# Autodesk Inventor assembly: しゃーし
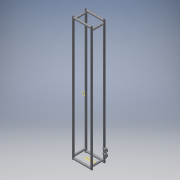
[picture p0: Inventor's stored thumbnail of the model, 180x180]
Saved by Autodesk Inventor 2018 (Build 220112000, 112)
## iProperties
Created: 2017-09-10
Part Number: しゃーし
Material: 一般
Document SubType Name: Assembly
Designer: Kenta
Author: Kenta
## Documents named in this file (7)
- C:\Users\Kenta\Documents\workspace\rbbr\cart\シャーシ\しゃーし.iam
- C:\Users\Kenta\Documents\workspace\rbbr\cart\シャーシ\横のパイプ.ipt
- C:\Users\Kenta\Documents\workspace\rbbr\cart\シャーシ\縦のパイプ.ipt
- C:\Users\Kenta\Documents\workspace\rbbr\cart\シャーシ\高さのパイプ.ipt
- C:\Users\Kenta\Documents\workspace\rbbr\cart\シャーシ\左右に飛び出すパイプ.ipt
- C:\Users\Kenta\Documents\workspace\rbbr\cart\シャーシ\14mmパイプ.ipt
- C:\Users\Kenta\Documents\workspace\rbbr\cart\シャーシ\hn1_14.ipt
## Components (17 placed, 6 different names)
1. 横のパイプ:1 — メイト:1, メイト:2, メイト:4, メイト:6, メイト:7, メイト:8, 角度:1
2. 縦のパイプ:1 — メイト:3, メイト:4, メイト:7, メイト:9, メイト:11, メイト:12, メイト:25, メイト:28, メイト:29, フラッシュ:3
3. 縦のパイプ:2 — メイト:5, メイト:6, メイト:8, メイト:10, メイト:21, メイト:23, メイト:27, メイト:30
4. 横のパイプ:2 — メイト:9, メイト:10, メイト:11
5. 高さのパイプ:1 — メイト:12, 角度:1, メイト:20, メイト:28
6. 横のパイプ:3
7. 縦のパイプ:3 — メイト:20, メイト:24, フラッシュ:3
8. 縦のパイプ:4 — メイト:22, メイト:26, メイト:31, メイト:33
9. 横のパイプ:4
10. 高さのパイプ:2 — メイト:24, メイト:25, メイト:29
11. 高さのパイプ:3 — メイト:23, メイト:26, メイト:30
12. 高さのパイプ:4 — メイト:21, メイト:22, メイト:27
13. 左右に飛び出すパイプ:1 — メイト:31, メイト:32, メイト:36
14. 14mmパイプ:1 — メイト:32, メイト:34, メイト:35, フラッシュ:4, メイト:37, フラッシュ:5
15. 左右に飛び出すパイプ:2 — メイト:33, メイト:34, メイト:38
16. hn1_14:1 — メイト:35, メイト:36, フラッシュ:4
17. hn1_14:2 — メイト:37, メイト:38, フラッシュ:5
## Relationships (44: Mate 38, Flush 5, Angle 1)
- フラッシュ:1 [Flush]
- メイト:1 [Mate]: 横のパイプ:1
- フラッシュ:2 [Flush]
- メイト:2 [Mate]: 横のパイプ:1
- メイト:3 [Mate]: 縦のパイプ:1
- メイト:4 [Mate]: 横のパイプ:1 ↔ 縦のパイプ:1
- メイト:5 [Mate]: 縦のパイプ:2
- メイト:6 [Mate]: 横のパイプ:1 ↔ 縦のパイプ:2
- メイト:7 [Mate] (-13.6 mm): 横のパイプ:1 ↔ 縦のパイプ:1
- メイト:8 [Mate] (-13.6 mm): 横のパイプ:1 ↔ 縦のパイプ:2
- メイト:9 [Mate]: 縦のパイプ:1 ↔ 横のパイプ:2
- メイト:10 [Mate]: 縦のパイプ:2 ↔ 横のパイプ:2
- メイト:11 [Mate] (-13.6 mm): 縦のパイプ:1 ↔ 横のパイプ:2
- メイト:12 [Mate]: 縦のパイプ:1 ↔ 高さのパイプ:1
- 角度:1 [Angle] (-90 deg): 横のパイプ:1 ↔ 高さのパイプ:1
- [Mate]: 横のパイプ:3 ↔ 縦のパイプ:3
- [Mate]: 横のパイプ:3 ↔ 縦のパイプ:4
- [Mate] (-13.6 mm): 横のパイプ:3 ↔ 縦のパイプ:3
- [Mate] (-13.6 mm): 横のパイプ:3 ↔ 縦のパイプ:4
- [Mate]: 縦のパイプ:3 ↔ 横のパイプ:4
- [Mate]: 縦のパイプ:4 ↔ 横のパイプ:4
- [Mate] (-13.6 mm): 縦のパイプ:3 ↔ 横のパイプ:4
- メイト:20 [Mate]: 高さのパイプ:1 ↔ 縦のパイプ:3
- メイト:21 [Mate]: 縦のパイプ:2 ↔ 高さのパイプ:4
- メイト:22 [Mate]: 縦のパイプ:4 ↔ 高さのパイプ:4
- メイト:23 [Mate]: 縦のパイプ:2 ↔ 高さのパイプ:3
- メイト:24 [Mate]: 縦のパイプ:3 ↔ 高さのパイプ:2
- メイト:25 [Mate]: 縦のパイプ:1 ↔ 高さのパイプ:2
- メイト:26 [Mate]: 縦のパイプ:4 ↔ 高さのパイプ:3
- メイト:27 [Mate] (-40.8 mm): 縦のパイプ:2 ↔ 高さのパイプ:4
- メイト:28 [Mate] (-40.8 mm): 縦のパイプ:1 ↔ 高さのパイプ:1
- メイト:29 [Mate] (-40.8 mm): 縦のパイプ:1 ↔ 高さのパイプ:2
- メイト:30 [Mate] (-40.8 mm): 縦のパイプ:2 ↔ 高さのパイプ:3
- フラッシュ:3 [Flush]: 縦のパイプ:1 ↔ 縦のパイプ:3
- メイト:31 [Mate]: 縦のパイプ:4 ↔ 左右に飛び出すパイプ:1
- メイト:32 [Mate]: 左右に飛び出すパイプ:1 ↔ 14mmパイプ:1
- メイト:33 [Mate]: 縦のパイプ:4 ↔ 左右に飛び出すパイプ:2
- メイト:34 [Mate]: 14mmパイプ:1 ↔ 左右に飛び出すパイプ:2
- メイト:35 [Mate]: 14mmパイプ:1 ↔ hn1_14:1
- メイト:36 [Mate]: 左右に飛び出すパイプ:1 ↔ hn1_14:1
- フラッシュ:4 [Flush]: 14mmパイプ:1 ↔ hn1_14:1
- メイト:37 [Mate]: 14mmパイプ:1 ↔ hn1_14:2
- メイト:38 [Mate]: 左右に飛び出すパイプ:2 ↔ hn1_14:2
- フラッシュ:5 [Flush]: 14mmパイプ:1 ↔ hn1_14:2
## Named parameters: d21_d13 = 0 mm, d22_d15 = 0 mm, d23_d16 = -13.6 mm, d24_d8 = 0 mm, d25_d10 = 0 mm, d26_d11 = -13.6 mm, d27_d12 = -13.6 mm
